# Autodesk Inventor assembly: cone_gopro_assembly
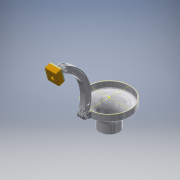
[picture p0: Inventor's stored thumbnail of the model, 180x180]
Saved by Autodesk Inventor 2019 (Build 230136000, 136)
## iProperties
Created: 2019-02-05
Part Number: cone_gopro_assembly
Document SubType Name: Assembly
Designer: jmc
Author: jmc
## Documents named in this file (6)
- C:\Users\l0086\Desktop\Models\CatFeeder\JarCone\version3\cone_gopro_assembly.iam
- C:\Users\l0086\Desktop\Models\CatFeeder\JarCone\version2\cono_nuevo.ipt
- C:\Users\l0086\Desktop\Models\3party\Gopro\Mount\mount_clean.ipt
- C:\Users\l0086\Desktop\Models\3party\Gopro\CurvedArm.ipt
- C:\Users\l0086\Desktop\Models\3party\raspberry case hdmi\case_with_gopro_mount_Shrinkwrap_1.ipt
- C:\Users\l0086\Desktop\Models\3party\raspberry case hdmi\hdmicase_bottom_clean.ipt
## Components (5 placed, 5 different names)
1. cono_nuevo:1
2. mount_clean:1 — Cylindrical:1
3. CurvedArm:1 — Cylindrical:1, Cylindrical:2
4. case_with_gopro_mount_Shrinkwrap_1:1 — Cylindrical:2, Rigid:1
5. hdmicase_bottom_clean:1 — Rigid:1
## Relationships (3: CylindricalJoint 2, WeldJoint 1)
- Cylindrical:1: mount_clean:1 ↔ CurvedArm:1
- Cylindrical:2: CurvedArm:1 ↔ case_with_gopro_mount_Shrinkwrap_1:1
- Rigid:1 [WeldJoint]: case_with_gopro_mount_Shrinkwrap_1:1 ↔ hdmicase_bottom_clean:1
